# Autodesk Inventor assembly: Муфта в сборе
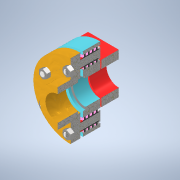
[picture p0: Inventor's stored thumbnail of the model, 180x180]
Saved by Autodesk Inventor 2021 (Build 250183000, 183)
## iProperties
Created: 2023-04-15
Part Number: Муфта в сборе
Document SubType Name: Assembly
Designer: gdevc
Author: gdevc
## Documents named in this file (11)
- C:\Users\gdevc\OneDrive\Рабочий стол\Курсач\DetaliMashine\Новая папка\Муфта в сборе.iam
- C:\Users\gdevc\OneDrive\Рабочий стол\Курсач\DetaliMashine\Новая папка\Муфта_Корпус.ipt
- C:\Users\gdevc\OneDrive\Рабочий стол\Курсач\DetaliMashine\Новая папка\Палец_ребрышко.ipt
- C:\Users\gdevc\OneDrive\Рабочий стол\Курсач\DetaliMashine\Новая папка\ANSI B 18.2.4.1 M - M10 x 1,5Style 1.ipt
- C:\Users\gdevc\OneDrive\Рабочий стол\Курсач\DetaliMashine\Новая папка\Демфер пальца.ipt
- C:\Users\gdevc\OneDrive\Рабочий стол\Курсач\DetaliMashine\Новая папка\Проставка.ipt
- C:\Users\gdevc\OneDrive\Рабочий стол\Курсач\DetaliMashine\Новая папка\Винт A.M10-6gx18 ГОСТ 17473-80.ipt
- C:\Users\gdevc\OneDrive\Рабочий стол\Курсач\DetaliMashine\Новая папка\Штрифт.ipt
- C:\Users\gdevc\OneDrive\Рабочий стол\Курсач\DetaliMashine\Новая папка\Втулка_Штрифта.ipt
- C:\Users\gdevc\OneDrive\Рабочий стол\Курсач\DetaliMashine\Новая папка\Штрифт_MIR.ipt
- C:\Users\gdevc\OneDrive\Рабочий стол\Курсач\DetaliMashine\Новая папка\Втулка_Штрифта_MIR.ipt
## Components (31 placed, 10 different names)
1. Муфта_Корпус:1 — Совмещение:1, Совмещение:2, Совмещение:4, Совмещение:9, Совмещение:10, Совмещение:11, Совмещение:15, Совмещение:16
2. Винт A.M10-6gx18 ГОСТ 17473-80:1 — Совмещение:9, Совмещение:10, Угол:3
3. Штрифт:1 — Совмещение:11, Совмещение:12
4. Втулка_Штрифта:1 — Совмещение:12
5. Винт A.M10-6gx18 ГОСТ 17473-80:2 — Угол:4, Совмещение:14, Совмещение:15, Совмещение:16
6. Штрифт_MIR:1 — Совмещение:13
7. Втулка_Штрифта_MIR:1 — Совмещение:13, Совмещение:14
8. Демфер пальца:1 — Совмещение:5, Совмещение:6, Совмещение:7, Совмещение:8
9. Палец_ребрышко:1 — Совмещение:1, Совмещение:2, Совмещение:3, Угол:1, Совмещение:5, Совмещение:6
10. ANSI B 18.2.4.1 M - M10 x 1,5Style 1:1 — Совмещение:3, Угол:1, Угол:2, Совмещение:4
11. Демфер пальца:2
12. Палец_ребрышко:2
13. ANSI B 18.2.4.1 M - M10 x 1,5Style 1:2
14. Демфер пальца:3
15. Палец_ребрышко:3
16. ANSI B 18.2.4.1 M - M10 x 1,5Style 1:3
17. Демфер пальца:4
18. Палец_ребрышко:4
19. ANSI B 18.2.4.1 M - M10 x 1,5Style 1:4
20. Демфер пальца:5
21. Палец_ребрышко:5
22. ANSI B 18.2.4.1 M - M10 x 1,5Style 1:5
23. Демфер пальца:6
24. Палец_ребрышко:6
25. ANSI B 18.2.4.1 M - M10 x 1,5Style 1:6
26. Проставка:1 — Совмещение:7, Совмещение:8
27. Проставка:2
28. Проставка:3
29. Проставка:4
30. Проставка:5
31. Проставка:6
## Component patterns: (6 elements, first: Демфер пальца:1 + Палец_ребрышко:1 + ANSI B 18.2.4.1 M - M10 x 1,5Style 1:1), (6 elements, first: Проставка:1)
## Relationships (20: Mate 16, Angle 4)
- Совмещение:1 [Mate]: Муфта_Корпус:1 ↔ Палец_ребрышко:1
- Совмещение:2 [Mate]: Муфта_Корпус:1 ↔ Палец_ребрышко:1
- Совмещение:3 [Mate]: Палец_ребрышко:1 ↔ ANSI B 18.2.4.1 M - M10 x 1,5Style 1:1
- Угол:1 [Angle] (0 deg): Палец_ребрышко:1 ↔ ANSI B 18.2.4.1 M - M10 x 1,5Style 1:1
- Угол:2 [Angle] (0 deg): ANSI B 18.2.4.1 M - M10 x 1,5Style 1:1
- Совмещение:4 [Mate]: Муфта_Корпус:1 ↔ ANSI B 18.2.4.1 M - M10 x 1,5Style 1:1
- Совмещение:5 [Mate]: Демфер пальца:1 ↔ Палец_ребрышко:1
- Совмещение:6 [Mate]: Демфер пальца:1 ↔ Палец_ребрышко:1
- Совмещение:7 [Mate]: Демфер пальца:1 ↔ Проставка:1
- Совмещение:8 [Mate]: Демфер пальца:1 ↔ Проставка:1
- Совмещение:9 [Mate]: Муфта_Корпус:1 ↔ Винт A.M10-6gx18 ГОСТ 17473-80:1
- Совмещение:10 [Mate]: Муфта_Корпус:1 ↔ Винт A.M10-6gx18 ГОСТ 17473-80:1
- Совмещение:11 [Mate]: Муфта_Корпус:1 ↔ Штрифт:1
- Совмещение:12 [Mate]: Штрифт:1 ↔ Втулка_Штрифта:1
- Совмещение:13 [Mate]: Штрифт_MIR:1 ↔ Втулка_Штрифта_MIR:1
- Угол:3 [Angle] (0 deg): Винт A.M10-6gx18 ГОСТ 17473-80:1
- Угол:4 [Angle] (0 deg): Винт A.M10-6gx18 ГОСТ 17473-80:2
- Совмещение:14 [Mate]: Винт A.M10-6gx18 ГОСТ 17473-80:2 ↔ Втулка_Штрифта_MIR:1
- Совмещение:15 [Mate]: Муфта_Корпус:1 ↔ Винт A.M10-6gx18 ГОСТ 17473-80:2
- Совмещение:16 [Mate]: Муфта_Корпус:1 ↔ Винт A.M10-6gx18 ГОСТ 17473-80:2
